# Autodesk Inventor assembly: arm4
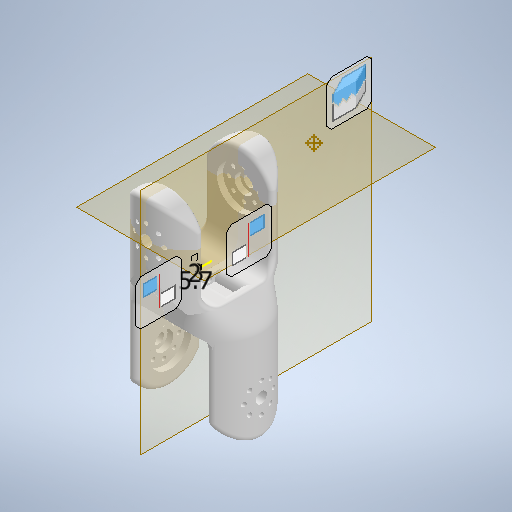
[picture p0: Inventor's stored thumbnail of the model, 512x512]
Saved by Autodesk Inventor 2026.1 (Build 301233020, 233B)
## iProperties
Created: 2025-09-20
Part Number: arm4
Document SubType Name: Assembly
Designer: wlgns
Author: wlgns
## Documents named in this file (3)
- C:\Users\wlgns\Desktop\Assistant Arm Project\ASSISTANT ARM MODEL\ASSISTANT ARM_origin\arm4.iam
- C:\Users\wlgns\Desktop\Assistant Arm Project\ASSISTANT ARM MODEL\ASSISTANT ARM_origin\end arm_1 - R.ipt
- C:\Users\wlgns\Desktop\Assistant Arm Project\ASSISTANT ARM MODEL\ASSISTANT ARM_origin\end arm_1 - L.ipt
## Components (2 placed, 2 different names)
1. end arm_1 - R:1 — 메이트:1, 메이트:2, 강체:1, 메이트:4
2. end arm_1 - L:1 — 메이트:2, 강체:1, 메이트:3
## Relationships (5: Mate 4, WeldJoint 1)
- 메이트:1 [Mate]: end arm_1 - R:1
- 메이트:2 [Mate]: end arm_1 - R:1 ↔ end arm_1 - L:1
- 강체:1 [WeldJoint]: end arm_1 - R:1 ↔ end arm_1 - L:1
- 메이트:3 [Mate]: end arm_1 - L:1
- 메이트:4 [Mate]: end arm_1 - R:1
